# Autodesk Inventor assembly: Hook Assembly
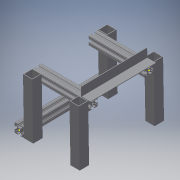
[picture p0: Inventor's stored thumbnail of the model, 180x180]
Saved by Autodesk Inventor 2018 (Build 220112000, 112)
## iProperties
Created: 2020-01-24
Part Number: Hook Assembly
Document SubType Name: Assembly
Designer: s-2513398
Author: s-2513398
## Documents named in this file (6)
- \\studenthome\students\S-2513398\GitHub\2020CAD\Climber Files\Parts\Hook Assembly .iam
- \\studenthome\students\S-2513398\GitHub\2020CAD\Climber Files\Parts\1010.ipt
- \\studenthome\students\S-2513398\GitHub\2020CAD\Climber Files\Parts\Hook 1st 1x1.ipt
- \\studenthome\students\S-2513398\GitHub\2020CAD\Climber Files\Parts\Hook 2nd 1x1.ipt
- \\studenthome\students\S-2513398\GitHub\2020CAD\Climber Files\Parts\Hook base.ipt
- \\studenthome\students\S-2513398\GitHub\2020CAD\Climber Files\Parts\Hook7in L Channel.ipt
## Components (8 placed, 5 different names)
1. 1010:1 — Mate:8, Flush:1, Flush:2, Flush:3, Flush:4, Mate:9, Mate:14
2. Hook 1st 1x1:1 — Mate:8, Flush:1, Flush:2
3. Hook 2nd 1x1:1 — Flush:3, Flush:4, Mate:9, Mate:12, Flush:7
4. Hook base:1 — Mate:12, Flush:7, Mate:17, Flush:12
5. 1010:2 — Mate:7, Flush:8, Mate:15, Flush:9, Flush:10, Flush:11, Mate:16
6. Hook 1st 1x1:2 — Flush:8, Mate:15, Flush:9
7. Hook 2nd 1x1:2 — Flush:10, Flush:11, Mate:16, Mate:17, Flush:12
8. Hook7in L Channel:1 — Mate:7, Mate:14
## Relationships (18: Flush 10, Mate 8)
- Mate:7: 1010:2 ↔ Hook7in L Channel:1
- Mate:8: 1010:1 ↔ Hook 1st 1x1:1
- Flush:1: 1010:1 ↔ Hook 1st 1x1:1
- Flush:2: 1010:1 ↔ Hook 1st 1x1:1
- Flush:3: 1010:1 ↔ Hook 2nd 1x1:1
- Flush:4: 1010:1 ↔ Hook 2nd 1x1:1
- Mate:9: 1010:1 ↔ Hook 2nd 1x1:1
- Mate:12: Hook 2nd 1x1:1 ↔ Hook base:1
- Flush:7: Hook 2nd 1x1:1 ↔ Hook base:1
- Mate:14: 1010:1 ↔ Hook7in L Channel:1
- Flush:8: 1010:2 ↔ Hook 1st 1x1:2
- Mate:15: 1010:2 ↔ Hook 1st 1x1:2
- Flush:9: 1010:2 ↔ Hook 1st 1x1:2
- Flush:10: 1010:2 ↔ Hook 2nd 1x1:2
- Flush:11: 1010:2 ↔ Hook 2nd 1x1:2
- Mate:16: 1010:2 ↔ Hook 2nd 1x1:2
- Mate:17: Hook base:1 ↔ Hook 2nd 1x1:2
- Flush:12: Hook base:1 ↔ Hook 2nd 1x1:2
